# Autodesk Inventor assembly: Recessed Wheels V1.0
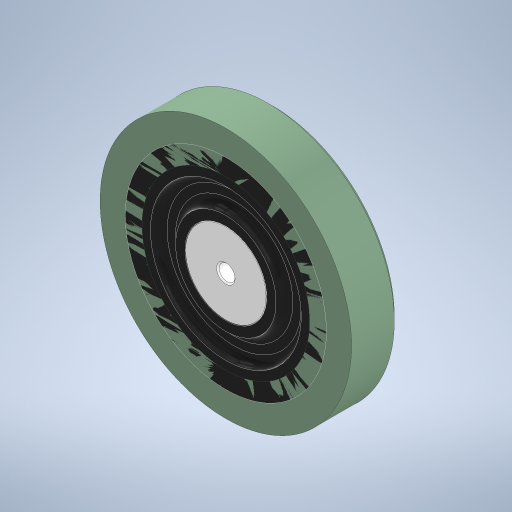
[picture p0: Inventor's stored thumbnail of the model, 512x512]
Saved by Autodesk Inventor 2023.2 (Build 272271000, 271)
## iProperties
Created: 2023-02-06
Part Number: Recessed Wheels V1.0
Document SubType Name: Assembly
Designer: Nathan Cai
Mass: 37.0779 g
Surface Area: 111.741 cm^2
Volume: 16.017 cm^3
Density: 2.31491 g/cm^3
Author: Nathan Cai
## Documents named in this file (4)
- C:\Users\Nathan Cai\Documents\Inventor\Moon Cake V0.16\Custom Wheel V2.0\Recessed Wheels V2.0.iam
- C:\Users\Nathan Cai\Documents\Inventor\Moon Cake V0.16\Custom Wheel V2.0\Tire Hub.ipt
- C:\Users\Nathan Cai\Documents\Inventor\Moon Cake V0.16\Custom Wheel V2.0\Tire.ipt
- C:\Users\Nathan Cai\Documents\Inventor\Moon Cake V0.16\Custom Wheel V2.0\T40_Hub_With_Retainer\T40_Hub_With_Retainer.iam
## Components (3 placed, 3 different names)
1. Tire Hub:1 — Flush:5, Mate:5, Mate:6, Mate:7, Flush:6
2. Tire:1 — Flush:5, Mate:5
3. T40_Hub_With_Retainer:1 [sub-assembly] — Mate:6, Mate:7, Flush:6
## Relationships (5: Mate 3, Flush 2)
- Flush:5: Tire Hub:1 ↔ Tire:1
- Mate:5: Tire Hub:1 ↔ Tire:1
- Mate:6: Tire Hub:1 ↔ T40_Hub_With_Retainer:1
- Mate:7 (0.0635 mm): Tire Hub:1 ↔ T40_Hub_With_Retainer:1
- Flush:6: Tire Hub:1 ↔ T40_Hub_With_Retainer:1
